# Autodesk Inventor assembly: Assembly2
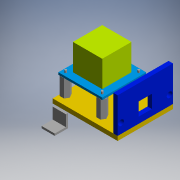
[picture p0: Inventor's stored thumbnail of the model, 180x180]
Saved by Autodesk Inventor 2016 (Build 200138000, 138)
## iProperties
Created: 2018-01-17
Part Number: Assembly2
Document SubType Name: Assembly
Designer: student
Author: student
## Documents named in this file (8)
- C:\Users\student\Documents\Assembly2.iam
- C:\Users\student\Documents\Part2.ipt
- C:\Users\student\Documents\Axis  plotter\axis plotter motor timing pulley.ipt
- C:\Users\student\Documents\Part3.ipt
- C:\Users\student\Documents\Part9.ipt
- C:\Users\student\Documents\Part14.ipt
- C:\Users\student\Documents\Part15.ipt
- C:\Users\student\Documents\Part16.ipt
## Components (10 placed, 7 different names)
1. Part2:1 — Insert:1, Angle:3, Mate:1, Mate:2, Angle:5, Angle:10
2. axis plotter motor timing pulley:1 — Insert:1
3. Part3:1 — Mate:1, Mate:2, Rigid:1, Rigid:4, Angle:4, Flush:2, Rigid:5, Rigid:6
4. Part9:1 — Rigid:1
5. Part9:3 — Rigid:4
6. Part9:4 — Rigid:5
7. Part9:5 — Rigid:6, Flush:3
8. Part14:1 — Flush:3, Flush:4
9. Part15:1 — Flush:4
10. Part16:1
## Relationships (17: Angle 6, WeldJoint 4, Flush 4, Mate 2, Insert 1)
- Insert:1: Part2:1 ↔ axis plotter motor timing pulley:1
- Angle:3 (180 deg): Part2:1
- Mate:1: Part2:1 ↔ Part3:1
- Mate:2: Part2:1 ↔ Part3:1
- Rigid:1 [WeldJoint]: Part3:1 ↔ Part9:1
- Rigid:4 [WeldJoint]: Part3:1 ↔ Part9:3
- Angle:4 (0 deg): Part3:1
- Flush:1 (-56 mm)
- Angle:5 (0 deg): Part2:1
- Flush:2 (30 mm): Part3:1
- Angle:8 (0 deg)
- Angle:9 (0 deg)
- Rigid:5 [WeldJoint]: Part3:1 ↔ Part9:4
- Rigid:6 [WeldJoint]: Part3:1 ↔ Part9:5
- Flush:3: Part9:5 ↔ Part14:1
- Flush:4: Part14:1 ↔ Part15:1
- Angle:10 (0 deg): Part2:1
